# Autodesk Inventor assembly: Krabicka
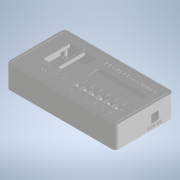
[picture p0: Inventor's stored thumbnail of the model, 180x180]
Saved by Autodesk Inventor 2021.2 (Build 252289000, 289)
## iProperties
Created: 2022-05-06
Part Number: Krabicka
Document SubType Name: Assembly
Designer: herman
Author: herman
## Documents named in this file (3)
- C:\Users\Herman\ownCloud\Prace\Kicad\PromProg\Krabicka\Krabicka.iam
- C:\Users\Herman\ownCloud\Prace\Kicad\PromProg\Krabicka\bottom.ipt
- C:\Users\Herman\ownCloud\Prace\Kicad\PromProg\Krabicka\top.ipt
## Components (2 placed, 2 different names)
1. bottom:1 — Stejný směr:1, Stejný směr:2, Proti sobě:1
2. top:1 — Stejný směr:1, Stejný směr:2, Proti sobě:1
## Relationships (3: Flush 2, Mate 1)
- Stejný směr:1 [Flush]: bottom:1 ↔ top:1
- Stejný směr:2 [Flush]: bottom:1 ↔ top:1
- Proti sobě:1 [Mate]: bottom:1 ↔ top:1
